# Autodesk Inventor assembly: cutout
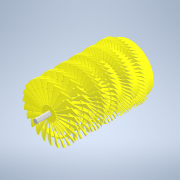
[picture p0: Inventor's stored thumbnail of the model, 180x180]
Saved by Autodesk Inventor 2021.2 (Build 252289000, 289)
## iProperties
Created: 2021-05-16
Part Number: cutout
Document SubType Name: Assembly
Designer: Ryan
Author: Ryan
## Documents named in this file (8)
- C:\Users\Ryan\Documents\EDD\__NewCompressor\cutout.iam
- C:\Users\Ryan\Documents\EDD\__NewCompressor\Axle.ipt
- C:\Users\Ryan\Documents\EDD\__NewCompressor\Rotor.24.1.0.ipt
- C:\Users\Ryan\Documents\EDD\__NewCompressor\Rotor.24.1.4.ipt
- C:\Users\Ryan\Documents\EDD\__NewCompressor\Rotor.36.1.8.ipt
- C:\Users\Ryan\Documents\EDD\__NewCompressor\Rotor.36.2.2.ipt
- C:\Users\Ryan\Documents\EDD\__NewCompressor\Rotor.48.2.6.ipt
- C:\Users\Ryan\Documents\EDD\__NewCompressor\Rotor.48.3.0.ipt
## Components (7 placed, 7 different names)
1. Axle:1 — Insert:14
2. Rotor.24.1.0:1 — Insert:14, Insert:15
3. Rotor.24.1.4:1 — Insert:15, Insert:16
4. Rotor.36.1.8:1 — Insert:16, Insert:17
5. Rotor.36.2.2:1 — Insert:17, Insert:18
6. Rotor.48.2.6:1 — Insert:18, Insert:19
7. Rotor.48.3.0:1 — Insert:19
## Relationships (6: Insert 6)
- Insert:14 (25.4 mm): Axle:1 ↔ Rotor.24.1.0:1
- Insert:15: Rotor.24.1.0:1 ↔ Rotor.24.1.4:1
- Insert:16: Rotor.24.1.4:1 ↔ Rotor.36.1.8:1
- Insert:17: Rotor.36.1.8:1 ↔ Rotor.36.2.2:1
- Insert:18: Rotor.36.2.2:1 ↔ Rotor.48.2.6:1
- Insert:19: Rotor.48.2.6:1 ↔ Rotor.48.3.0:1
